# Autodesk Inventor assembly: ParticleLauncherwCollector
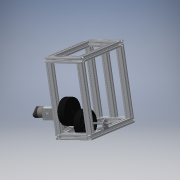
[picture p0: Inventor's stored thumbnail of the model, 180x180]
Saved by Autodesk Inventor 2016 (Build 200138000, 138)
## iProperties
Created: 2016-10-12
Part Number: ParticleLauncherwCollector
Document SubType Name: Assembly
Designer: Delta
Author: Delta
## Documents named in this file (15)
- C:\Robotics\CAD\2016-17_CAD\ParticleLauncher2.0.iam
- C:\Robotics\CAD\COTSParts\Actobotics\555 parts\555116.ipt
- C:\Robotics\CAD\COTSParts\Actobotics\am-3102NeveRest20 (1).ipt
- C:\Robotics\CAD\COTSParts\Actobotics\634 parts\634088.ipt
- C:\Robotics\CAD\COTSParts\Wheels\4in Wheel Intergreated Hub 8mm Rev2.ipt
- C:\Robotics\CAD\COTSParts\Bearings - AndyMark\Bearing 250 ID 500 OD flanged.ipt
- C:\Robotics\CAD\COTSParts\Actobotics\545 parts\545400.ipt
- C:\Robotics\CAD\COTSParts\Bosch Extrusion\6mm block nut M4.ipt
- C:\Robotics\CAD\COTSParts\Bosch Extrusion\Bosch 20x20 - 4.5 Part.Shoot.ipt
- C:\Robotics\CAD\COTSParts\Bosch Extrusion\Gusset 20x20 w screws.ipt
- C:\Robotics\CAD\COTSParts\Bosch Extrusion\Bosch 20x20 13 in.ipt
- C:\Robotics\CAD\COTSParts\Actobotics\585 parts\585422.ipt
- C:\Robotics\CAD\COTSParts\Bosch Extrusion\Bosch 20x20 9 real.ipt
- C:\Robotics\CAD\COTSParts\Bosch Extrusion\Bosch 20x20 5.5.ipt
- C:\Robotics\CAD\COTSParts\Bosch Extrusion\Bosch 20x20 7.675.ipt
## Components (33 placed, 14 different names)
1. 555116:1 — Insert:15, Insert:38, Insert:39
2. am-3102NeveRest20 (1):1 — Insert:15, Insert:34
3. 634088:1 — Mate:84, Mate:85, Flush:8, Mate:86, Mate:87
4. 4in Wheel Intergreated Hub 8mm Rev2:1 — Mate:86, Mate:87, Mate:88
5. 4in Wheel Intergreated Hub 8mm Rev2:2 — Insert:34
6. Bearing 250 ID 500 OD flanged:2 — Mate:77, Mate:78, Mate:85
7. Bearing 250 ID 500 OD flanged:3 — Mate:82, Mate:83, Mate:84
8. 545400:1 — Mate:80, Mate:81, Mate:82, Mate:83, Flush:8, Mate:89
9. 545400:2 — Mate:74, Mate:76, Mate:77, Mate:78, Insert:35
10. 6mm block nut M4:4 — Mate:69, Mate:80
11. 6mm block nut M4:5 — Mate:68, Mate:70, Mate:81
12. 6mm block nut M4:6 — Mate:71, Mate:72, Mate:74, Mate:76
13. 6mm block nut M4:7 — Insert:35, Mate:106
14. Bosch 20x20 - 4.5 Part.Shoot:1 — Mate:30, Mate:31, Mate:34, Mate:35, Mate:45, Flush:3, Flush:4, Flush:5, Flush:6, Mate:48, Mate:89
15. Gusset 20x20 w screws:1 — Mate:30, Mate:31, Mate:53
16. Gusset 20x20 w screws:2 — Mate:34, Mate:35, Mate:52
17. Bosch 20x20 13 in:1 — Flush:5, Flush:6, Mate:48, Mate:53, Mate:56, Mate:57, Mate:67, Mate:68, Mate:69, Mate:70, Mate:88, Mate:105, Flush:34, Flush:35, Flush:36
18. Bosch 20x20 13 in:2 — Mate:45, Flush:3, Flush:4, Mate:52, Mate:61, Mate:64, Mate:65, Flush:7, Mate:71, Mate:72, Mate:106
19. Bosch 20x20 - 4.5 Part.Shoot:2 — Mate:62, Mate:63, Mate:66, Mate:67, Flush:7
20. Gusset 20x20 w screws:3 — Mate:56, Mate:57, Mate:66
21. Gusset 20x20 w screws:4 — Mate:61, Mate:62, Mate:63, Mate:64, Mate:65
22. Bosch 20x20 9 real:1 — Flush:25, Mate:104, Flush:32, Flush:33, Mate:105, Flush:34, Flush:35, Mate:107, Mate:108, Mate:109
23. Bosch 20x20 9 real:2 — Mate:101, Flush:29, Flush:30
24. Bosch 20x20 9 real:3 — Mate:102, Flush:31, Mate:103
25. Bosch 20x20 9 real:4 — Mate:97, Flush:20, Flush:21
26. Bosch 20x20 9 real:5 — Mate:96, Flush:18, Flush:19, Mate:103
27. Bosch 20x20 5.5:1 — Mate:97, Flush:20, Flush:21, Mate:98, Flush:22, Flush:23, Mate:99, Flush:24, Flush:26, Mate:104, Flush:32, Flush:33
28. Bosch 20x20 5.5:2 — Mate:96, Flush:18, Flush:19, Mate:100, Flush:27, Flush:28, Mate:101, Flush:29, Flush:30, Mate:102, Flush:31
29. Bosch 20x20 7.675:1 — Mate:99, Flush:24, Flush:25, Flush:26, Mate:100, Flush:27, Flush:28
30. Bosch 20x20 7.675:2 — Mate:98, Flush:22, Flush:23
31. 585422:1 — Insert:36, Insert:37, Insert:38, Insert:39
32. 6mm block nut M4:8 — Mate:107, Flush:36, Insert:36
33. 6mm block nut M4:9 — Mate:108, Mate:109, Insert:37
## Relationships (82: Mate 50, Flush 25, Insert 7)
- Insert:15 (-17.78 mm): 555116:1 ↔ am-3102NeveRest20 (1):1
- Insert:34 (-10.16 mm): am-3102NeveRest20 (1):1 ↔ 4in Wheel Intergreated Hub 8mm Rev2:2
- Mate:30: Bosch 20x20 - 4.5 Part.Shoot:1 ↔ Gusset 20x20 w screws:1
- Mate:31: Bosch 20x20 - 4.5 Part.Shoot:1 ↔ Gusset 20x20 w screws:1
- Mate:34: Bosch 20x20 - 4.5 Part.Shoot:1 ↔ Gusset 20x20 w screws:2
- Mate:35: Bosch 20x20 - 4.5 Part.Shoot:1 ↔ Gusset 20x20 w screws:2
- Mate:45: Bosch 20x20 - 4.5 Part.Shoot:1 ↔ Bosch 20x20 13 in:2
- Flush:3: Bosch 20x20 - 4.5 Part.Shoot:1 ↔ Bosch 20x20 13 in:2
- Flush:4: Bosch 20x20 - 4.5 Part.Shoot:1 ↔ Bosch 20x20 13 in:2
- Flush:5: Bosch 20x20 - 4.5 Part.Shoot:1 ↔ Bosch 20x20 13 in:1
- Flush:6: Bosch 20x20 - 4.5 Part.Shoot:1 ↔ Bosch 20x20 13 in:1
- Mate:48: Bosch 20x20 - 4.5 Part.Shoot:1 ↔ Bosch 20x20 13 in:1
- Mate:52: Gusset 20x20 w screws:2 ↔ Bosch 20x20 13 in:2
- Mate:53: Gusset 20x20 w screws:1 ↔ Bosch 20x20 13 in:1
- Mate:56: Bosch 20x20 13 in:1 ↔ Gusset 20x20 w screws:3
- Mate:57: Bosch 20x20 13 in:1 ↔ Gusset 20x20 w screws:3
- Mate:61: Bosch 20x20 13 in:2 ↔ Gusset 20x20 w screws:4
- Mate:62: Bosch 20x20 - 4.5 Part.Shoot:2 ↔ Gusset 20x20 w screws:4
- Mate:63: Bosch 20x20 - 4.5 Part.Shoot:2 ↔ Gusset 20x20 w screws:4
- Mate:64: Bosch 20x20 13 in:2 ↔ Gusset 20x20 w screws:4
- Mate:65: Bosch 20x20 13 in:2 ↔ Gusset 20x20 w screws:4
- Mate:66: Bosch 20x20 - 4.5 Part.Shoot:2 ↔ Gusset 20x20 w screws:3
- Mate:67: Bosch 20x20 13 in:1 ↔ Bosch 20x20 - 4.5 Part.Shoot:2
- Flush:7: Bosch 20x20 13 in:2 ↔ Bosch 20x20 - 4.5 Part.Shoot:2
- Mate:68: 6mm block nut M4:5 ↔ Bosch 20x20 13 in:1
- Mate:69: 6mm block nut M4:4 ↔ Bosch 20x20 13 in:1
- Mate:70: 6mm block nut M4:5 ↔ Bosch 20x20 13 in:1
- Mate:71: 6mm block nut M4:6 ↔ Bosch 20x20 13 in:2
- Mate:72: 6mm block nut M4:6 ↔ Bosch 20x20 13 in:2
- Mate:74: 545400:2 ↔ 6mm block nut M4:6
- Mate:76: 545400:2 ↔ 6mm block nut M4:6
- Mate:77: Bearing 250 ID 500 OD flanged:2 ↔ 545400:2
- Mate:78: Bearing 250 ID 500 OD flanged:2 ↔ 545400:2
- Mate:80: 545400:1 ↔ 6mm block nut M4:4
- Mate:81: 545400:1 ↔ 6mm block nut M4:5
- Mate:82: Bearing 250 ID 500 OD flanged:3 ↔ 545400:1
- Mate:83: Bearing 250 ID 500 OD flanged:3 ↔ 545400:1
- Mate:84: 634088:1 ↔ Bearing 250 ID 500 OD flanged:3
- Mate:85: 634088:1 ↔ Bearing 250 ID 500 OD flanged:2
- Flush:8 (-25.4 mm): 634088:1 ↔ 545400:1
- Mate:86: 634088:1 ↔ 4in Wheel Intergreated Hub 8mm Rev2:1
- Mate:87: 634088:1 ↔ 4in Wheel Intergreated Hub 8mm Rev2:1
- Mate:88 (37.1475 mm): 4in Wheel Intergreated Hub 8mm Rev2:1 ↔ Bosch 20x20 13 in:1
- Mate:89 (38.1 mm): 545400:1 ↔ Bosch 20x20 - 4.5 Part.Shoot:1
- Mate:96: Bosch 20x20 9 real:5 ↔ Bosch 20x20 5.5:2
- Flush:18: Bosch 20x20 9 real:5 ↔ Bosch 20x20 5.5:2
- Flush:19: Bosch 20x20 9 real:5 ↔ Bosch 20x20 5.5:2
- Mate:97: Bosch 20x20 9 real:4 ↔ Bosch 20x20 5.5:1
- Flush:20: Bosch 20x20 9 real:4 ↔ Bosch 20x20 5.5:1
- Flush:21: Bosch 20x20 9 real:4 ↔ Bosch 20x20 5.5:1
- Mate:98: Bosch 20x20 5.5:1 ↔ Bosch 20x20 7.675:2
- Flush:22: Bosch 20x20 5.5:1 ↔ Bosch 20x20 7.675:2
- Flush:23: Bosch 20x20 5.5:1 ↔ Bosch 20x20 7.675:2
- Mate:99: Bosch 20x20 5.5:1 ↔ Bosch 20x20 7.675:1
- Flush:24: Bosch 20x20 5.5:1 ↔ Bosch 20x20 7.675:1
- Flush:25: Bosch 20x20 9 real:1 ↔ Bosch 20x20 7.675:1
- Flush:26: Bosch 20x20 5.5:1 ↔ Bosch 20x20 7.675:1
- Mate:100: Bosch 20x20 5.5:2 ↔ Bosch 20x20 7.675:1
- Flush:27: Bosch 20x20 5.5:2 ↔ Bosch 20x20 7.675:1
- Flush:28: Bosch 20x20 5.5:2 ↔ Bosch 20x20 7.675:1
- Mate:101: Bosch 20x20 9 real:2 ↔ Bosch 20x20 5.5:2
- Flush:29: Bosch 20x20 9 real:2 ↔ Bosch 20x20 5.5:2
- Flush:30: Bosch 20x20 9 real:2 ↔ Bosch 20x20 5.5:2
- Mate:102: Bosch 20x20 9 real:3 ↔ Bosch 20x20 5.5:2
- Flush:31: Bosch 20x20 9 real:3 ↔ Bosch 20x20 5.5:2
- Mate:103 (39.8526 mm): Bosch 20x20 9 real:3 ↔ Bosch 20x20 9 real:5
- Mate:104: Bosch 20x20 9 real:1 ↔ Bosch 20x20 5.5:1
- Flush:32: Bosch 20x20 9 real:1 ↔ Bosch 20x20 5.5:1
- Flush:33: Bosch 20x20 9 real:1 ↔ Bosch 20x20 5.5:1
- Mate:105: Bosch 20x20 13 in:1 ↔ Bosch 20x20 9 real:1
- Flush:34: Bosch 20x20 13 in:1 ↔ Bosch 20x20 9 real:1
- Flush:35: Bosch 20x20 13 in:1 ↔ Bosch 20x20 9 real:1
- Insert:35: 545400:2 ↔ 6mm block nut M4:7
- Mate:106: 6mm block nut M4:7 ↔ Bosch 20x20 13 in:2
- Mate:107: Bosch 20x20 9 real:1 ↔ 6mm block nut M4:8
- Mate:108: Bosch 20x20 9 real:1 ↔ 6mm block nut M4:9
- Mate:109: Bosch 20x20 9 real:1 ↔ 6mm block nut M4:9
- Flush:36 (78.74 mm): Bosch 20x20 13 in:1 ↔ 6mm block nut M4:8
- Insert:36: 585422:1 ↔ 6mm block nut M4:8
- Insert:37: 585422:1 ↔ 6mm block nut M4:9
- Insert:38: 555116:1 ↔ 585422:1
- Insert:39: 555116:1 ↔ 585422:1
